# Autodesk Inventor assembly: suport + senzor
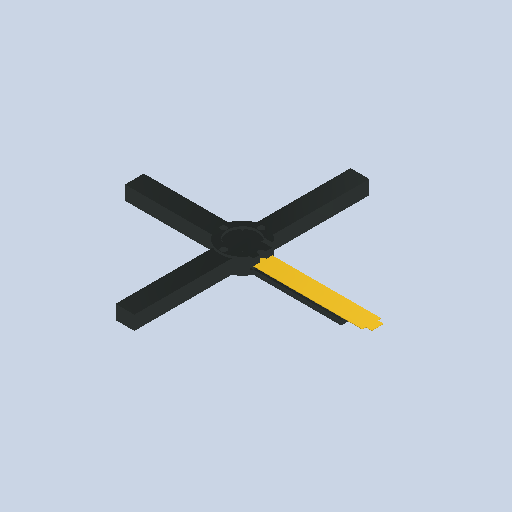
[picture p0: Inventor's stored thumbnail of the model, 512x512]
Saved by Autodesk Inventor 2022 (Build 260153000, 153)
## iProperties
Created: 2022-02-27
Part Number: suport + senzor
Document SubType Name: Assembly
Designer: Oana
Author: Oana
## Documents named in this file (3)
- D:\salvari\aplicatii-proiecte\infoeducatia 2022\proiectare\pat_scanare\suport + senzor.iam
- D:\salvari\aplicatii-proiecte\infoeducatia 2022\proiectare\pat_scanare\prindere senzor.ipt
- D:\salvari\aplicatii-proiecte\infoeducatia 2022\proiectare\piese\senzor presiune.ipt
## Components (2 placed, 2 different names)
1. prindere senzor:1 — Rotational:1
2. senzor presiune:1 — Rotational:1
## Relationships (1: RevoluteJoint 1)
- Rotational:1 [RevoluteJoint]: prindere senzor:1 ↔ senzor presiune:1
